# Autodesk Inventor assembly: ploter-plate
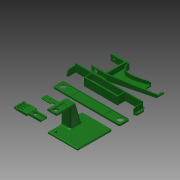
[picture p0: Inventor's stored thumbnail of the model, 180x180]
Saved by Autodesk Inventor 2013 (Build 170138000, 138)
## iProperties
Created: 2014-06-28
Part Number: ploter-plate
Document SubType Name: Assembly
Designer: Masta
Author: Masta
## Documents named in this file (7)
- D:\rysownik\3D models\ploter-plate.iam
- D:\rysownik\3D models\arm1.ipt
- D:\rysownik\3D models\arm1a.ipt
- D:\rysownik\3D models\arm2.ipt
- D:\rysownik\3D models\base.ipt
- D:\rysownik\3D models\hand1.ipt
- D:\rysownik\3D models\hand2.ipt
## Components (6 placed, 6 different names)
1. arm1:1 — Mate:1
2. arm1a:1 — Mate:2
3. arm2:1 — Mate:1
4. base:1 — Mate:3
5. hand1:1 — Mate:5
6. hand2:1 — Mate:4
## Relationships (6: Mate 6)
- Mate:1: arm1:1
- Mate:2: arm1a:1
- Mate:1: arm2:1
- Mate:3: base:1
- Mate:4: hand2:1
- Mate:5: hand1:1
